# Autodesk Inventor assembly: Сборка1
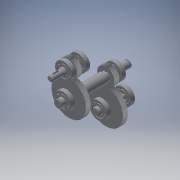
[picture p0: Inventor's stored thumbnail of the model, 180x180]
Saved by Autodesk Inventor 2018 (Build 220112000, 112)
## iProperties
Created: 2018-06-10
Part Number: Сборка1
Material: Типовые
Document SubType Name: Assembly
Designer: katya
Author: katya
## Documents named in this file (13)
- C:\Users\katya\Desktop\Новая папка (3)\Сборка1.iam
- C:\Users\katya\Desktop\Новая папка (3)\sborka\Вал 3.ipt
- C:\Users\katya\Desktop\Новая папка (3)\sborka\Вал 1.ipt
- C:\Users\katya\Desktop\Новая папка (3)\sborka\Колесо 1.ipt
- C:\Users\katya\Desktop\Новая папка (3)\sborka\Колесо 2.ipt
- C:\Users\katya\Desktop\Новая папка (3)\sborka\Подшипник 1.ipt
- C:\Users\katya\Desktop\Новая папка (3)\sborka\Подшипник 2.ipt
- C:\Users\katya\Desktop\Новая папка (3)\sborka\Подшипник 3.ipt
- C:\Users\katya\Desktop\Новая папка (3)\sborka\Подшипник 4.ipt
- C:\Users\katya\Desktop\Новая папка (3)\sborka\Подшипник 5.ipt
- C:\Users\katya\Desktop\Новая папка (3)\sborka\Подшипник 6.ipt
- C:\Users\katya\Desktop\Новая папка (3)\sborka\Шестерня 1.ipt
- C:\Users\katya\Desktop\Новая папка (3)\sborka\Шестерня 2.ipt
## Components (13 placed, 1 different names)
1. Деталь:1 — Совмещение:1, Совмещение:5, Совмещение:6, Совмещение:7, Совмещение:9
2. Деталь:2 — Совмещение:2, Совмещение:3, Совмещение:4
3. Деталь:5 — Совмещение:1, Заподлицо:1
4. Деталь:6 — Совмещение:8, Угол:1, Касательность:1, Заподлицо:2
5. Деталь:7 — Совмещение:3
6. Деталь:8 — Совмещение:4
7. Деталь:9 — Совмещение:6
8. Деталь:10 — Совмещение:7
9. Деталь:11 — Совмещение:10
10. Деталь:12 — Совмещение:11
11. Деталь:13 — Заподлицо:1, Совмещение:2
12. Деталь:14 — Совмещение:5, Касательность:1, Заподлицо:2
13. Деталь:15 — Совмещение:8, Угол:1, Совмещение:9, Совмещение:10, Совмещение:11
## Relationships (15: Mate 11, Flush 2, Angle 1, Tangent 1)
- Совмещение:1 [Mate]: Деталь:1 ↔ Деталь:5
- Заподлицо:1 [Flush]: Деталь:5 ↔ Деталь:13
- Совмещение:2 [Mate]: Деталь:2 ↔ Деталь:13
- Совмещение:3 [Mate]: Деталь:2 ↔ Деталь:7
- Совмещение:4 [Mate]: Деталь:2 ↔ Деталь:8
- Совмещение:5 [Mate]: Деталь:1 ↔ Деталь:14
- Совмещение:6 [Mate]: Деталь:1 ↔ Деталь:9
- Совмещение:7 [Mate]: Деталь:1 ↔ Деталь:10
- Совмещение:8 [Mate]: Деталь:6 ↔ Деталь:15
- Угол:1 [Angle] (0 deg): Деталь:6 ↔ Деталь:15
- Касательность:1 [Tangent]: Деталь:6 ↔ Деталь:14
- Совмещение:9 [Mate]: Деталь:1 ↔ Деталь:15
- Заподлицо:2 [Flush]: Деталь:6 ↔ Деталь:14
- Совмещение:10 [Mate]: Деталь:11 ↔ Деталь:15
- Совмещение:11 [Mate]: Деталь:12 ↔ Деталь:15
